# Autodesk Inventor assembly: LiquidPiston
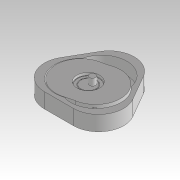
[picture p0: Inventor's stored thumbnail of the model, 180x180]
Saved by Autodesk Inventor 2020 (Build 240168000, 168)
## iProperties
Created: 2021-07-13
Part Number: LiquidPiston
Document SubType Name: Assembly
Designer: DDeGo
Author: DDeGo
## Documents named in this file (5)
- C:\Users\DDeGo\Documents\Drew\Projects\AirWankelEngine\cad\LiquidPiston V1\LiquidPiston.iam
- C:\Users\DDeGo\Documents\Drew\Projects\AirWankelEngine\cad\LiquidPiston V1\Housing.ipt
- C:\Users\DDeGo\Documents\Drew\Projects\AirWankelEngine\cad\LiquidPiston V1\Rotor.ipt
- C:\Users\DDeGo\Documents\Drew\Projects\AirWankelEngine\cad\hardware\6701 bearing.ipt
- C:\Users\DDeGo\Documents\Drew\Projects\AirWankelEngine\cad\LiquidPiston V1\Camshaft.ipt
## Components (4 placed, 4 different names)
1. Housing:1 — Flush:1, Flush:2, Flush:3, Mate:3, Mate:5
2. Rotor:1 — Mate:1, Mate:2, Mate:3, Rotation:1
3. 6701 bearing:1 — Mate:1, Mate:2, Flush:4, Mate:4
4. Camshaft:1 — Flush:4, Mate:4, Mate:5, Rotation:1
## Relationships (10: Mate 5, Flush 4, RelateRotation 1)
- Flush:1: Housing:1
- Flush:2: Housing:1
- Flush:3: Housing:1
- Mate:1: Rotor:1 ↔ 6701 bearing:1
- Mate:2: Rotor:1 ↔ 6701 bearing:1
- Mate:3: Housing:1 ↔ Rotor:1
- Flush:4: 6701 bearing:1 ↔ Camshaft:1
- Mate:4: 6701 bearing:1 ↔ Camshaft:1
- Mate:5: Housing:1 ↔ Camshaft:1
- Rotation:1 [RelateRotation] (2 ul): Rotor:1 ↔ Camshaft:1
